# Autodesk Inventor assembly: 21
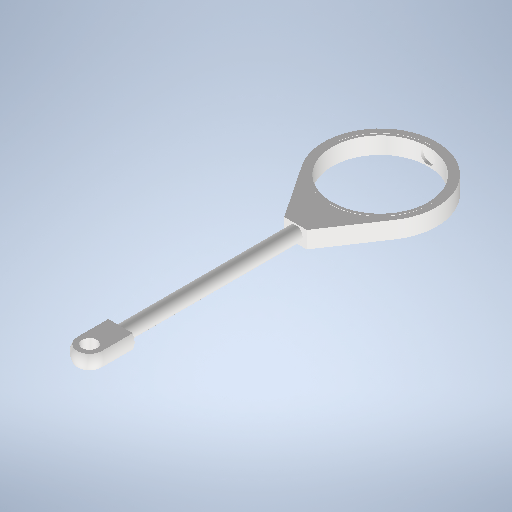
[picture p0: Inventor's stored thumbnail of the model, 512x512]
Saved by Autodesk Inventor 2025.1 (Build 291241000, 241)
## iProperties
Created: 2024-09-13
Part Number: 21
Document SubType Name: Assembly
Designer: ffogue
Author: ffogue
## Documents named in this file (4)
- C:\Users\ffogue\Documents\Inventor\Single cylinder Steam Engine\21.iam
- C:\Users\ffogue\Documents\Inventor\Single cylinder Steam Engine\21.1.ipt
- C:\Users\ffogue\Documents\Inventor\Single cylinder Steam Engine\21.ipt
- C:\Users\ffogue\Documents\Inventor\Single cylinder Steam Engine\21.2.ipt
## Components (3 placed, 3 different names)
1. 21.1:1 — Mate:1, Rotational:1
2. 21:1 — Mate:1, Rotational:1, Mate:2, Insert:1
3. 21.2:1 — Mate:2, Insert:1
## Relationships (4: Mate 2, RevoluteJoint 1, Insert 1)
- Mate:1: 21.1:1 ↔ 21:1
- Rotational:1 [RevoluteJoint]: 21.1:1 ↔ 21:1
- Mate:2: 21:1 ↔ 21.2:1
- Insert:1 (-4 mm): 21:1 ↔ 21.2:1
